# Autodesk Inventor assembly: Assembly mueble cajon gde
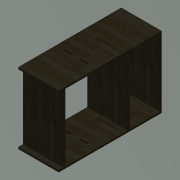
[picture p0: Inventor's stored thumbnail of the model, 180x180]
Saved by Autodesk Inventor 2015 (Build 190159000, 159)
## iProperties
Created: 2016-01-26
Part Number: Assembly mueble cajon gde
Document SubType Name: Assembly
Designer: iberopuebla
Author: iberopuebla
## Documents named in this file (4)
- H:\3d\Assembly mueble cajon gde.iam
- H:\3d\repisaa.ipt
- H:\3d\tapa laterales.ipt
- H:\3d\tapa sup.ipt
## Components (5 placed, 3 different names)
1. tapa laterales:1 — Mate:1, Flush:1, Mate:2, Flush:2, Flush:3, Flush:4, Mate:3, Mate:4, Flush:6, Mate:7, Mate:8
2. tapa sup:1 — Mate:1, Flush:1, Mate:2, Flush:2, Flush:3, Flush:8
3. repisaa:2 — Flush:6, Mate:7, Mate:8, Flush:7
4. tapa laterales:2 — Flush:7, Mate:9, Flush:8
5. repisaa:3 — Flush:4, Mate:3, Mate:4, Mate:9
## Relationships (14: Mate 7, Flush 7)
- Mate:1: tapa laterales:1 ↔ tapa sup:1
- Flush:1: tapa laterales:1 ↔ tapa sup:1
- Mate:2: tapa laterales:1 ↔ tapa sup:1
- Flush:2: tapa laterales:1 ↔ tapa sup:1
- Flush:3: tapa laterales:1 ↔ tapa sup:1
- Flush:4: tapa laterales:1 ↔ repisaa:3
- Mate:3: tapa laterales:1 ↔ repisaa:3
- Mate:4: tapa laterales:1 ↔ repisaa:3
- Flush:6: tapa laterales:1 ↔ repisaa:2
- Mate:7: tapa laterales:1 ↔ repisaa:2
- Mate:8: tapa laterales:1 ↔ repisaa:2
- Flush:7: repisaa:2 ↔ tapa laterales:2
- Mate:9: tapa laterales:2 ↔ repisaa:3
- Flush:8: tapa sup:1 ↔ tapa laterales:2
